# Autodesk Inventor assembly: FullV1
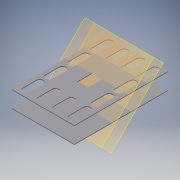
[picture p0: Inventor's stored thumbnail of the model, 180x180]
Saved by Autodesk Inventor 2019 (Build 230136000, 136)
## iProperties
Created: 2021-09-15
Part Number: FullV1
Document SubType Name: Assembly
Designer: timmy
Author: timmy
## Documents named in this file (5)
- S:\Inventor\RoboCatz\T-Shirt\FullV1.iam
- S:\Inventor\RoboCatz\T-Shirt\R-O-SideV1.ipt
- S:\Inventor\RoboCatz\T-Shirt\Top.ipt
- S:\Inventor\RoboCatz\T-Shirt\NamePlateV1.ipt
- S:\Inventor\RoboCatz\T-Shirt\BottomV1.ipt
## Components (6 placed, 4 different names)
1. R-O-SideV1:1 — Flush:1, Mate:1, Flush:2, Flush:9
2. Top:1 — Flush:1, Mate:1, Flush:2, Flush:3, Flush:4, Mate:2, Flush:5, Mate:3, Mate:6, Mate:7, Angle:1
3. R-O-SideV1:2 — Flush:3, Flush:4, Mate:2, Flush:6, Flush:7, Flush:8, Flush:11, Mate:4
4. NamePlateV1:1 — Flush:5, Flush:6, Flush:7, Flush:10
5. NamePlateV1:2 — Flush:8, Mate:3, Flush:9
6. BottomV1:1 — Flush:10, Flush:11, Mate:4, Mate:5
## Relationships (20: Flush 12, Mate 7, Angle 1)
- Flush:1: R-O-SideV1:1 ↔ Top:1
- Mate:1: R-O-SideV1:1 ↔ Top:1
- Flush:2: R-O-SideV1:1 ↔ Top:1
- Flush:3: Top:1 ↔ R-O-SideV1:2
- Flush:4: Top:1 ↔ R-O-SideV1:2
- Mate:2: Top:1 ↔ R-O-SideV1:2
- Flush:5: Top:1 ↔ NamePlateV1:1
- Flush:6: R-O-SideV1:2 ↔ NamePlateV1:1
- Flush:7: R-O-SideV1:2 ↔ NamePlateV1:1
- Flush:8: R-O-SideV1:2 ↔ NamePlateV1:2
- Mate:3: Top:1 ↔ NamePlateV1:2
- Flush:9: R-O-SideV1:1 ↔ NamePlateV1:2
- Flush:10: NamePlateV1:1 ↔ BottomV1:1
- Flush:11: R-O-SideV1:2 ↔ BottomV1:1
- Mate:4: R-O-SideV1:2 ↔ BottomV1:1
- Mate:5: BottomV1:1
- Mate:6: Top:1
- Mate:7: Top:1
- Angle:1 (0 deg): Top:1
- Flush:12 (-131.7625 mm)
